# Autodesk Inventor assembly: Case
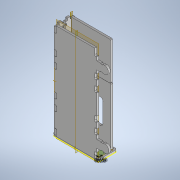
[picture p0: Inventor's stored thumbnail of the model, 180x180]
Saved by Autodesk Inventor 2020 (Build 240168000, 168)
## iProperties
Created: 2019-12-17
Part Number: Case
Document SubType Name: Assembly
Designer: erwin
Author: erwin
## Documents named in this file (8)
- D:\GitHub\ElCheapoAIS-nmea\case\Wooden Multicase\prototype\Case.iam
- D:\GitHub\ElCheapoAIS-nmea\case\Wooden Multicase\prototype\interior.ipt
- D:\GitHub\ElCheapoAIS-nmea\case\Wooden Multicase\prototype\cover.ipt
- D:\GitHub\ElCheapoAIS-nmea\case\Wooden Multicase\prototype\parameters.ipt
- D:\GitHub\ElCheapoAIS-nmea\case\Wooden Multicase\side_side.ipt
- D:\GitHub\ElCheapoAIS-nmea\case\Wooden Multicase\cover_components.ipt
- D:\GitHub\ElCheapoAIS-nmea\case\Wooden Multicase\cover_wires.ipt
- D:\GitHub\ElCheapoAIS-nmea\case\Wooden Multicase\dxf\new_side_bottom.ipt
## Components (8 placed, 7 different names)
1. interior:1 — Flush:1, Flush:2, Flush:8, Flush:9
2. cover:1 — Flush:1, Flush:2, Flush:10, Mate:1, Flush:12, Flush:13
3. parameters:1
4. side_side:1 — Flush:8, Flush:9
5. side_side:2 — Flush:10, Mate:1, Flush:11
6. cover_components:1 — Flush:11
7. cover_wires:1
8. new_side_bottom:1 — Flush:12, Flush:13
## Relationships (9: Flush 8, Mate 1)
- Flush:1: interior:1 ↔ cover:1
- Flush:2: interior:1 ↔ cover:1
- Flush:8: interior:1 ↔ side_side:1
- Flush:9: interior:1 ↔ side_side:1
- Flush:10: cover:1 ↔ side_side:2
- Mate:1: cover:1 ↔ side_side:2
- Flush:11: side_side:2 ↔ cover_components:1
- Flush:12: cover:1 ↔ new_side_bottom:1
- Flush:13: cover:1 ↔ new_side_bottom:1
